# Autodesk Inventor assembly: Rebel_LED_on_CP01_M
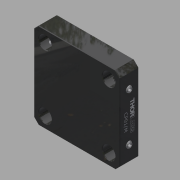
[picture p0: Inventor's stored thumbnail of the model, 180x180]
Saved by Autodesk Inventor 2018 (Build 220112000, 112)
## iProperties
Created: 2018-11-07
Part Number: Rebel_LED_on_CP01_M
Document SubType Name: Assembly
Designer: Robert Campbell
Author: Robert Campbell
## Documents named in this file (3)
- \\Mac\Home\Dropbox (UCL - SWC)\work\WorkDocs\MF_BenchOptics\CAD_files\Rebel_LED_on_CP01_M.iam
- \\Mac\Home\Dropbox (UCL - SWC)\work\WorkDocs\MF_BenchOptics\CAD_files\Rebel_Star_LED_CAD.ipt
- \\Mac\Home\Dropbox (UCL - SWC)\work\WorkDocs\MF_BenchOptics\CAD_files\CP01_M-Solidworks.ipt
## Components (2 placed, 2 different names)
1. Rebel_Star_LED_CAD:1 — Mate:1, Flush:1, Mate:2
2. CP01_M-Solidworks:1 — Mate:1, Flush:1, Mate:2
## Relationships (3: Mate 2, Flush 1)
- Mate:1: Rebel_Star_LED_CAD:1 ↔ CP01_M-Solidworks:1
- Flush:1 (10 mm): Rebel_Star_LED_CAD:1 ↔ CP01_M-Solidworks:1
- Mate:2 (-9 mm): Rebel_Star_LED_CAD:1 ↔ CP01_M-Solidworks:1
